# Autodesk Inventor assembly: Klapp-Baugruppe
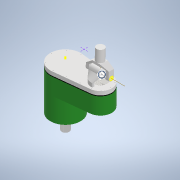
[picture p0: Inventor's stored thumbnail of the model, 180x180]
Saved by Autodesk Inventor 2021 (Build 250183000, 183)
## iProperties
Created: 2021-01-12
Part Number: Klapp-Baugruppe
Document SubType Name: Assembly
Designer: Jaro Machnow
Author: Jaro Machnow
## Documents named in this file (15)
- C:\Users\Jaro Machnow\Documents\Vault\Gruppen\Gruppe 2\Entwurf\Amphibienfahrzeug\Wechsel zwischen Land und Wasser\Wechselmechanik\Klappmechanismus2\Klapp-Baugruppe.iam
- C:\Users\Jaro Machnow\Documents\Vault\Gruppen\Gruppe 2\Entwurf\Amphibienfahrzeug\Wechsel zwischen Land und Wasser\Wechselmechanik\Klappmechanismus\Klapphülle.ipt
- C:\Users\Jaro Machnow\Documents\Vault\Gruppen\Gruppe 2\Entwurf\Amphibienfahrzeug\Wechsel zwischen Land und Wasser\Wechselmechanik\Klappmechanismus\Welle1_zur_Karosserie.ipt
- C:\Users\Jaro Machnow\Documents\Vault\Gruppen\Gruppe 2\Entwurf\Amphibienfahrzeug\Wechsel zwischen Land und Wasser\Wechselmechanik\Klappmechanismus\Kraftübertragung mit Keilriemen.iam
- C:\Users\Jaro Machnow\Documents\Vault\Gruppen\Gruppe 2\Entwurf\Amphibienfahrzeug\Wechsel zwischen Land und Wasser\Wechselmechanik\Klappmechanismus\Lager1.iam
- C:\Users\Jaro Machnow\Documents\Vault\Gruppen\Gruppe 2\Entwurf\Amphibienfahrzeug\Wechsel zwischen Land und Wasser\Wechselmechanik\Klappmechanismus\Keilverbindung1.iam
- C:\Users\Jaro Machnow\Documents\Vault\Gruppen\Gruppe 2\Entwurf\Amphibienfahrzeug\Wechsel zwischen Land und Wasser\Wechselmechanik\Klappmechanismus\Dichtungsgummi.ipt
- C:\Users\Jaro Machnow\Documents\Vault\Gruppen\Gruppe 2\Entwurf\Amphibienfahrzeug\Betrieb an Land\Lenkung\Lenkung_Baugruppe.iam
- C:\Users\Jaro Machnow\Documents\Vault\Gruppen\Gruppe 2\Entwurf\Amphibienfahrzeug\Wechsel zwischen Land und Wasser\Wechselmechanik\Klappmechanismus2\Abdeckung_für_Lenkung.ipt
- C:\Users\Jaro Machnow\Documents\Vault\Gruppen\Gruppe 2\Entwurf\Amphibienfahrzeug\Wechsel zwischen Land und Wasser\Wechselmechanik\Klappmechanismus2\Klapp-Baugruppe\Konstruktions-Assistent\Keilverbindung4.iam
- C:\Users\Jaro Machnow\Documents\Vault\Gruppen\Gruppe 2\Entwurf\Amphibienfahrzeug\Betrieb an Land\Lenkung\Lenkteil_zum_Rad.ipt
- C:\Users\Jaro Machnow\Documents\Vault\Gruppen\Gruppe 2\Entwurf\Amphibienfahrzeug\Wechsel zwischen Land und Wasser\Wechselmechanik\Klappmechanismus2\Welle3.ipt
- C:\Users\Jaro Machnow\Documents\Vault\Gruppen\Gruppe 2\Entwurf\Amphibienfahrzeug\Wechsel zwischen Land und Wasser\Wechselmechanik\Klappmechanismus2\Welle2.ipt
- C:\Users\Jaro Machnow\Documents\Vault\Gruppen\Gruppe 2\Entwurf\Amphibienfahrzeug\Wechsel zwischen Land und Wasser\Wechselmechanik\Klappmechanismus2\Klapp-Baugruppe\Konstruktions-Assistent\Keilverbindung5.iam
- C:\Users\Jaro Machnow\Documents\Vault\Gruppen\Gruppe 2\Entwurf\Amphibienfahrzeug\Wechsel zwischen Land und Wasser\Wechselmechanik\Klappmechanismus2\Klapp-Baugruppe\Konstruktions-Assistent\Keilverbindung6.iam
## Components (17 placed, 9 different names)
1. Welle:1 — Passend:1, Passend:5, Fluchtend:6, Passend:10, Passend:11, Passend:12, Winkel:2, Passend:46, Fluchtend:15, Winkel:24, Passend:69
2. Kraftübertragung mit Keilriemen:1 [sub-assembly] — Passend:1, Passend:10, Winkel:2, Passend:61, Passend:66, Winkel:21
3. Lager:1 [sub-assembly] — Passend:5, Fluchtend:6, Passend:21
4. Lager:2 [sub-assembly] — Passend:64, Passend:65
5. Lager:3 [sub-assembly] — Passend:11, Passend:12
6. Keilverbindung:1 [sub-assembly] — Fluchtend:15, Winkel:24, Passend:69
7. Lager:4 [sub-assembly] — Passend:62, Passend:63
8. Klapphülle:1 — Passend:21, Passend:22, Passend:23, Passend:24, Passend:33, Passend:34, Passend:46
9. Dichtungsgummi:1 — Passend:22, Passend:23, Passend:24, Passend:32
10. Lenkung_Baugruppe:1 [sub-assembly] — Passend:56, Winkel:19, Winkel:23
11. Abdeckung_für_Lenkung:1 — Passend:32, Passend:33, Passend:34, Passend:55
12. Lenkteil_zum_Rad:1 — Passend:58, Passend:59, Passend:60
13. Welle:1 — Passend:55, Passend:56, Fluchtend:12, Winkel:18, Passend:57, Winkel:19, Passend:58, Passend:59, Passend:60
14. Keilverbindung:4 [sub-assembly] — Fluchtend:12, Winkel:18, Passend:57
15. Welle:1 — Passend:61, Passend:62, Passend:63, Passend:64, Passend:65, Passend:66, Fluchtend:13, Winkel:20, Passend:67, Winkel:21, Fluchtend:14, Winkel:22, Passend:68, Winkel:23
16. Keilverbindung:5 [sub-assembly] — Fluchtend:13, Winkel:20, Passend:67
17. Keilverbindung:6 [sub-assembly] — Fluchtend:14, Winkel:22, Passend:68
## Relationships (41: Mate 28, Angle 8, Flush 5)
- Passend:1 [Mate]: Welle:1 ↔ Kraftübertragung mit Keilriemen:1
- Passend:5 [Mate]: Welle:1 ↔ Lager:1
- Fluchtend:6 [Flush]: Welle:1 ↔ Lager:1
- Passend:10 [Mate]: Welle:1 ↔ Kraftübertragung mit Keilriemen:1
- Passend:11 [Mate]: Welle:1 ↔ Lager:3
- Passend:12 [Mate]: Welle:1 ↔ Lager:3
- Winkel:2 [Angle] (174.2383 deg): Welle:1 ↔ Kraftübertragung mit Keilriemen:1
- Passend:21 [Mate]: Lager:1 ↔ Klapphülle:1
- Passend:22 [Mate]: Klapphülle:1 ↔ Dichtungsgummi:1
- Passend:23 [Mate]: Klapphülle:1 ↔ Dichtungsgummi:1
- Passend:24 [Mate]: Klapphülle:1 ↔ Dichtungsgummi:1
- Passend:32 [Mate]: Dichtungsgummi:1 ↔ Abdeckung_für_Lenkung:1
- Passend:33 [Mate]: Klapphülle:1 ↔ Abdeckung_für_Lenkung:1
- Passend:34 [Mate]: Klapphülle:1 ↔ Abdeckung_für_Lenkung:1
- Passend:46 [Mate] (0.064 mm): Welle:1 ↔ Klapphülle:1
- Passend:55 [Mate]: Abdeckung_für_Lenkung:1 ↔ Welle:1
- Passend:56 [Mate]: Lenkung_Baugruppe:1 ↔ Welle:1
- Fluchtend:12 [Flush] (0.371 mm): Welle:1 ↔ Keilverbindung:4
- Winkel:18 [Angle] (0 deg): Welle:1 ↔ Keilverbindung:4
- Passend:57 [Mate]: Welle:1 ↔ Keilverbindung:4
- Winkel:19 [Angle] (173.4856 deg): Lenkung_Baugruppe:1 ↔ Welle:1
- Passend:58 [Mate]: Lenkteil_zum_Rad:1 ↔ Welle:1
- Passend:59 [Mate]: Lenkteil_zum_Rad:1 ↔ Welle:1
- Passend:60 [Mate]: Lenkteil_zum_Rad:1 ↔ Welle:1
- Passend:61 [Mate]: Kraftübertragung mit Keilriemen:1 ↔ Welle:1
- Passend:62 [Mate]: Lager:4 ↔ Welle:1
- Passend:63 [Mate]: Lager:4 ↔ Welle:1
- Passend:64 [Mate]: Lager:2 ↔ Welle:1
- Passend:65 [Mate]: Lager:2 ↔ Welle:1
- Passend:66 [Mate]: Kraftübertragung mit Keilriemen:1 ↔ Welle:1
- Fluchtend:13 [Flush] (6.7781 mm): Welle:1 ↔ Keilverbindung:5
- Winkel:20 [Angle] (0 deg): Welle:1 ↔ Keilverbindung:5
- Passend:67 [Mate]: Welle:1 ↔ Keilverbindung:5
- Winkel:21 [Angle] (141.9438 deg): Kraftübertragung mit Keilriemen:1 ↔ Welle:1
- Fluchtend:14 [Flush] (0.0883 mm): Welle:1 ↔ Keilverbindung:6
- Winkel:22 [Angle] (0 deg): Welle:1 ↔ Keilverbindung:6
- Passend:68 [Mate]: Welle:1 ↔ Keilverbindung:6
- Winkel:23 [Angle] (15.1609 deg): Lenkung_Baugruppe:1 ↔ Welle:1
- Fluchtend:15 [Flush] (1.0188 mm): Welle:1 ↔ Keilverbindung:1
- Winkel:24 [Angle] (0 deg): Welle:1 ↔ Keilverbindung:1
- Passend:69 [Mate]: Welle:1 ↔ Keilverbindung:1
